# Autodesk Inventor assembly: Assembly Station with parts
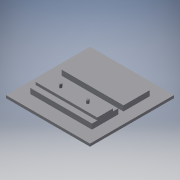
[picture p0: Inventor's stored thumbnail of the model, 180x180]
Saved by Autodesk Inventor 2019.4 (Build 234330000, 330)
## iProperties
Created: 2020-11-11
Part Number: Assembly Station with parts
Document SubType Name: Assembly
Designer: caleb
Author: caleb
## Documents named in this file (4)
- C:\Users\cfang\Desktop\CAD\TFPX\glue spreader jig\Assembly Station with parts.iam
- C:\Users\cfang\Desktop\CAD\TFPX\glue spreader jig\Assembly Station.ipt
- C:\Users\cfang\Downloads\8472A190_PRESS-FIT LOCATING PIN.ipt
- C:\Users\cfang\Downloads\8472A110_PRESS-FIT LOCATING PIN.ipt
## Components (3 placed, 3 different names)
1. Assembly Station:1 — Mate:1, Mate:2
2. 8472A190_PRESS-FIT LOCATING PIN:1 — Mate:1
3. 8472A110_PRESS-FIT LOCATING PIN:1 — Mate:2
## Relationships (2: Mate 2)
- Mate:1: Assembly Station:1 ↔ 8472A190_PRESS-FIT LOCATING PIN:1
- Mate:2: Assembly Station:1 ↔ 8472A110_PRESS-FIT LOCATING PIN:1
